# Autodesk Inventor assembly: leg_B_01
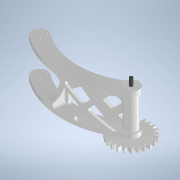
[picture p0: Inventor's stored thumbnail of the model, 180x180]
Saved by Autodesk Inventor 2020.2 (Build 242310000, 310)
## iProperties
Created: 2020-11-22
Part Number: leg_B_01
Document SubType Name: Assembly
Designer: mazzo
Author: mazzo
## Documents named in this file (4)
- D:\Documenti\università\Progetto Meccanica dei Robot\assembled in urdf\leg_B_01.iam
- D:\Documenti\università\Progetto Meccanica dei Robot\meccanica\parti autodesk\V6\V6 Luca\barra_filettata_inferiore.ipt
- D:\Documenti\università\Progetto Meccanica dei Robot\meccanica\parti autodesk\V6\V6 Luca\gamba1.ipt
- D:\Documenti\università\Progetto Meccanica dei Robot\meccanica\parti autodesk\V6\V6 Luca\Ingranaggio cilindrico esterno.ipt
## Components (3 placed, 3 different names)
1. barra_filettata_inferiore:1 — Coincidente:1, Allineato:2
2. gamba1:1 — Coincidente:3, Allineato:1, Coincidente:4, Coincidente:5, Allineato:2, Coincidente:6
3. Ingranaggio cilindrico1:1 — Coincidente:2, Coincidente:4, Coincidente:5
## Relationships (8: Mate 6, Flush 2)
- Coincidente:1 [Mate]: barra_filettata_inferiore:1
- Coincidente:2 [Mate]: Ingranaggio cilindrico1:1
- Coincidente:3 [Mate]: gamba1:1
- Allineato:1 [Flush]: gamba1:1
- Coincidente:4 [Mate]: gamba1:1 ↔ Ingranaggio cilindrico1:1
- Coincidente:5 [Mate]: gamba1:1 ↔ Ingranaggio cilindrico1:1
- Allineato:2 [Flush] (10 mm): barra_filettata_inferiore:1 ↔ gamba1:1
- Coincidente:6 [Mate]: gamba1:1
